# Autodesk Inventor assembly: LEG_PROTOTYPE_R1
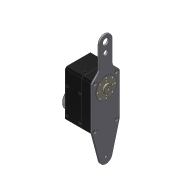
[picture p0: Inventor's stored thumbnail of the model, 180x180]
Saved by Autodesk Inventor 2019.4 (Build 234330000, 330)
## iProperties
Created: 2019-12-01
Part Number: LEG_PROTOTYPE_R1
Material: 一般
Document SubType Name: Assembly
Designer: y6tada
Author: y6tada
## Documents named in this file (3)
- C:\Workspace\Yuni9\Inventor\Asm\LEG_UNIT\LEG_PROTOTYPE_R1.iam
- C:\Workspace\Yuni9\Inventor\Libs\DYNAMIXEL\XM540\XM540_NO_BACK.iam
- C:\Workspace\Yuni9\Inventor\Asm\HEAD_CAMERA_UNIT\UPPER_LEG_BASE.ipt
## Components (2 placed, 2 different names)
1. XM540_NO_BACK:1 [sub-assembly] — フラッシュ:1, フラッシュ:2, フラッシュ:3, フラッシュ:4
2. UPPER_LEG_BASE:1 — フラッシュ:4, フラッシュ:5, フラッシュ:6
## Relationships (6: Flush 6)
- フラッシュ:1 [Flush] (75 mm): XM540_NO_BACK:1
- フラッシュ:2 [Flush]: XM540_NO_BACK:1
- フラッシュ:3 [Flush]: XM540_NO_BACK:1
- フラッシュ:4 [Flush]: XM540_NO_BACK:1 ↔ UPPER_LEG_BASE:1
- フラッシュ:5 [Flush]: UPPER_LEG_BASE:1
- フラッシュ:6 [Flush]: UPPER_LEG_BASE:1
